# Autodesk Inventor assembly: !Ramp
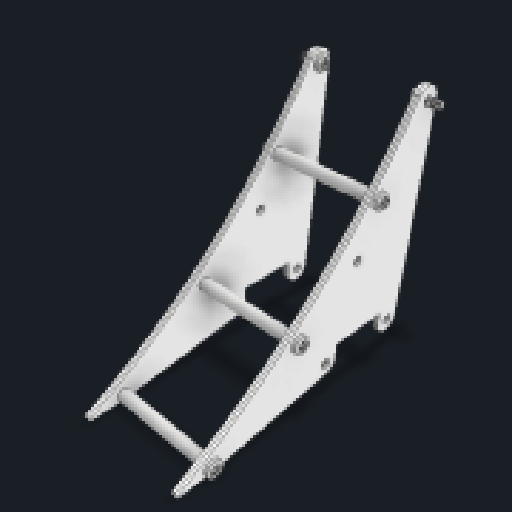
[picture p0: Inventor's stored thumbnail of the model, 512x512]
Saved by Autodesk Inventor 2025.1 (Build 291241000, 241)
## iProperties
Created: 2024-11-12
Part Number: !Ramp
Document SubType Name: Assembly
Designer: avere
Author: avere
## Documents named in this file (4)
- C:\Users\avere\VEX\High Stakes\CAD\V3\Chassis\Ramp\!Ramp.iam
- C:\Users\avere\VEX\High Stakes\CAD\V3\Chassis\Ramp\Custom Parts\Ramp.ipt
- C:\Users\avere\VEX\High Stakes\CAD\ROBOPROS-CAD-Inventor\Structure\Nylon Standoff Rounded\Nylon Standoff 2.000.ipt
- C:\Users\avere\VEX\High Stakes\CAD\ROBOPROS-CAD-Inventor\Structure\Hardware\Screw Nylon - Pan Head\NScrew Pan Head Threaded .375.ipt
## Components (15 placed, 3 different names)
1. Ramp:1 — Insert:3, Mate:4, Insert:7, Insert:8
2. Ramp:2 — Insert:2, Insert:3, Mate:4, Insert:4, Insert:5, Insert:10
3. Ramp:3 — Mate:1, Tangent:1, Mate:2, Insert:1, Mate:3, Insert:2, Insert:11, Insert:14
4. Ramp:4 — Insert:1, Mate:3, Insert:6, Insert:9, Angle:1
5. Nylon Standoff 2.000:1 — Insert:4
6. Nylon Standoff 2.000:2 — Insert:5
7. NScrew Pan Head Threaded .375:1 — Insert:7
8. NScrew Pan Head Threaded .375:2 — Insert:6
9. NScrew Pan Head Threaded .375:3 — Insert:8
10. NScrew Pan Head Threaded .375:4 — Insert:9
11. NScrew Pan Head Threaded .375:5 — Insert:11
12. NScrew Pan Head Threaded .375:6 — Insert:10
13. Nylon Standoff 2.000:3 — Insert:12, Insert:13, Insert:14
14. NScrew Pan Head Threaded .375:7 — Insert:13
15. NScrew Pan Head Threaded .375:8 — Insert:12
## Relationships (20: Insert 14, Mate 4, Tangent 1, Angle 1)
- Mate:1 (25.4 mm): Ramp:3
- Tangent:1: Ramp:3
- Mate:2: Ramp:3
- Insert:1: Ramp:3 ↔ Ramp:4
- Mate:3: Ramp:3 ↔ Ramp:4
- Insert:2 (50.8 mm): Ramp:2 ↔ Ramp:3
- Insert:3: Ramp:1 ↔ Ramp:2
- Mate:4: Ramp:1 ↔ Ramp:2
- Insert:4: Ramp:2 ↔ Nylon Standoff 2.000:1
- Insert:5: Ramp:2 ↔ Nylon Standoff 2.000:2
- Insert:6: Ramp:4 ↔ NScrew Pan Head Threaded .375:2
- Insert:7: Ramp:1 ↔ NScrew Pan Head Threaded .375:1
- Insert:8: Ramp:1 ↔ NScrew Pan Head Threaded .375:3
- Insert:9: Ramp:4 ↔ NScrew Pan Head Threaded .375:4
- Angle:1 (180 deg): Ramp:4
- Insert:10: Ramp:2 ↔ NScrew Pan Head Threaded .375:6
- Insert:11: Ramp:3 ↔ NScrew Pan Head Threaded .375:5
- Insert:12 (3.175 mm): Nylon Standoff 2.000:3 ↔ NScrew Pan Head Threaded .375:8
- Insert:13 (3.175 mm): Nylon Standoff 2.000:3 ↔ NScrew Pan Head Threaded .375:7
- Insert:14: Ramp:3 ↔ Nylon Standoff 2.000:3
